# Autodesk Inventor assembly: colimadores2
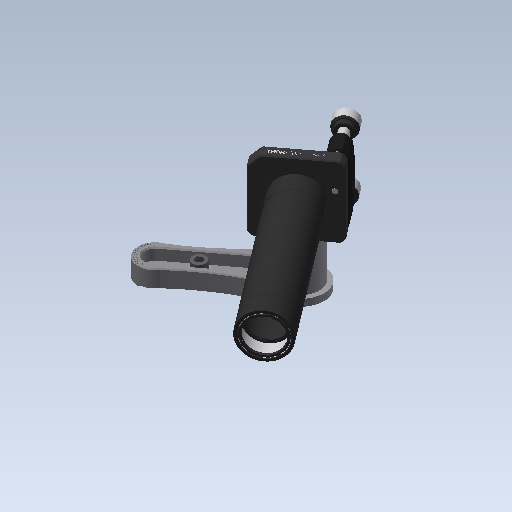
[picture p0: Inventor's stored thumbnail of the model, 512x512]
Saved by Autodesk Inventor 2020 (Build 240168000, 168)
## iProperties
Created: 2016-10-06
Part Number: colimadores2
Document SubType Name: Assembly
Designer: i7
Author: i7
## Documents named in this file (7)
- C:\LAFriOC\diseños\sistema de vacío\Óptica para la MOT\Colimadores para MOT\colimador pequeño.iam
- C:\LAFriOC\diseños\sistema de vacío\Óptica para la MOT\Colimadores para MOT\KS1T-kinematic mounts.ipt
- C:\LAFriOC\diseños\sistema de vacío\Óptica para la MOT\Colimadores para MOT\SM1L40-lens tube.ipt
- C:\LAFriOC\diseños\sistema de vacío\Óptica para la MOT\Colimadores para MOT\SM1L05.ipt
- C:\LAFriOC\diseños\sistema de vacío\Óptica para la MOT\Colimadores para MOT\SM1FCA-FC-APC fiber adapter.ipt
- C:\LAFriOC\diseños\sistema de vacío\Óptica para la MOT\Colimadores para MOT\CF175C-clamping.ipt
- C:\LAFriOC\diseños\sistema de vacío\Óptica para la MOT\Colimadores para MOT\small-post.ipt
## Components (7 placed, 6 different names)
1. KS1T-kinematic mounts:1 — De rotación:1, De rotación:4, Rígido:1
2. SM1L40-lens tube:1 — De rotación:1, De rotación:2
3. SM1L05:1 — De rotación:2
4. SM1L05:2 — De rotación:3, De rotación:4
5. SM1FCA-FC-APC fiber adapter:1 — De rotación:3
6. CF175C-clamping:1 — De rotación:5
7. small-post:1 — Rígido:1, De rotación:5
## Relationships (6: RevoluteJoint 5, WeldJoint 1)
- De rotación:1 [RevoluteJoint]: KS1T-kinematic mounts:1 ↔ SM1L40-lens tube:1
- De rotación:2 [RevoluteJoint]: SM1L40-lens tube:1 ↔ SM1L05:1
- De rotación:3 [RevoluteJoint]: SM1L05:2 ↔ SM1FCA-FC-APC fiber adapter:1
- De rotación:4 [RevoluteJoint]: KS1T-kinematic mounts:1 ↔ SM1L05:2
- Rígido:1 [WeldJoint]: KS1T-kinematic mounts:1 ↔ small-post:1
- De rotación:5 [RevoluteJoint]: CF175C-clamping:1 ↔ small-post:1
